# Autodesk Inventor assembly: AASTRC case
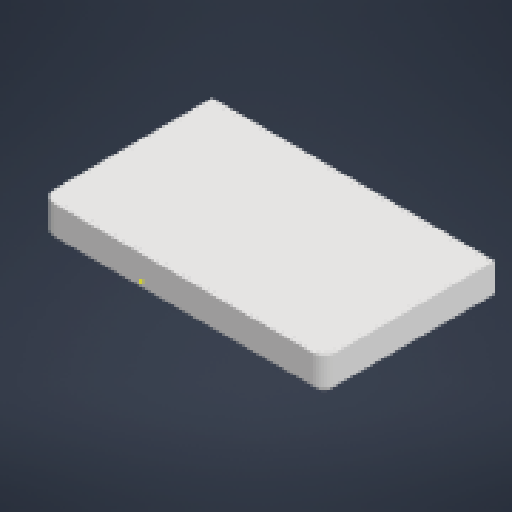
[picture p0: Inventor's stored thumbnail of the model, 512x512]
Saved by Autodesk Inventor 2024 (Build 280153000, 153)
## iProperties
Created: 2023-07-16
Part Number: AASTRC case
Document SubType Name: Assembly
Designer: 6gioc
Author: 6gioc
## Documents named in this file (6)
- C:\Users\wodyd\Downloads\AAST\PART\AAST Remote Controler\AASTRC case.iam
- C:\Users\wodyd\Downloads\AAST\PART\AAST Remote Controler\AASTRC Bottom case.ipt
- C:\Users\wodyd\Downloads\AAST\PART\AAST Remote Controler\AASTRC Bottom case cover.ipt
- C:\Users\wodyd\Downloads\AAST\PART\AAST Remote Controler\AASTRC Middle case cover assembly.iam
- C:\Users\wodyd\Downloads\AAST\PART\AAST Remote Controler\AASTRC Top case cover.iam
- C:\Users\wodyd\Downloads\AAST\PART\AAST Remote Controler\apple logo light module.iam
## Components (5 placed, 5 different names)
1. AASTRC Bottom case:1 — 강체:1, 강체:2, 강체:3, 강체:4
2. AASTRC Bottom case cover:1 — 강체:1
3. AASTRC Middle case cover assembly:1 [sub-assembly] — 강체:2
4. AASTRC Top case cover assemble:1 [sub-assembly] — 강체:3
5. apple logo light module:1 [sub-assembly] — 강체:4
## Relationships (4: WeldJoint 4)
- 강체:1 [WeldJoint]: AASTRC Bottom case:1 ↔ AASTRC Bottom case cover:1
- 강체:2 [WeldJoint]: AASTRC Bottom case:1 ↔ AASTRC Middle case cover assembly:1
- 강체:3 [WeldJoint]: AASTRC Bottom case:1 ↔ AASTRC Top case cover assemble:1
- 강체:4 [WeldJoint]: AASTRC Bottom case:1 ↔ apple logo light module:1
